# Autodesk Inventor assembly: Hex Shaft Assembly
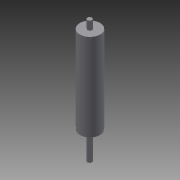
[picture p0: Inventor's stored thumbnail of the model, 180x180]
Saved by Autodesk Inventor 2015 (Build 190159000, 159)
## iProperties
Created: 2015-02-04
Part Number: Hex Shaft Assembly
Document SubType Name: Assembly
Designer: kaurdha17
Author: kaurdha17
## Documents named in this file (4)
- H:\Hex Shaft Assembly.iam
- H:\Part1.ipt
- H:\Part2.ipt
- H:\Part3.ipt
## Components (4 placed, 3 different names)
1. Part1:1 — Insert:1, Flush:1, Mate:1
2. Part2:1 — Insert:1, Insert:2
3. Part3:1 — Flush:1, Mate:1
4. Part1:2 — Insert:2
## Relationships (4: Insert 2, Flush 1, Mate 1)
- Insert:1: Part1:1 ↔ Part2:1
- Flush:1 (-25.4 mm): Part1:1 ↔ Part3:1
- Mate:1: Part1:1 ↔ Part3:1
- Insert:2: Part2:1 ↔ Part1:2
